# Autodesk Inventor assembly: Zespół1
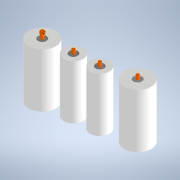
[picture p0: Inventor's stored thumbnail of the model, 180x180]
Saved by Autodesk Inventor 2022 (Build 260153000, 153)
## iProperties
Created: 2023-04-25
Part Number: Zespół1
Document SubType Name: Assembly
Designer: nosal
Author: nosal
## Documents named in this file (6)
- C:\Users\nosal\OneDrive\Pulpit\projekty 3d\Inżynierka\Tasma2\Zespół1.iam
- C:\Users\nosal\OneDrive\Pulpit\projekty 3d\Inżynierka\Tasma2\wał_tylni2.ipt
- C:\Users\nosal\OneDrive\Pulpit\projekty 3d\Inżynierka\Tasma2\wały_sr.ipt
- C:\Users\nosal\OneDrive\Pulpit\projekty 3d\Inżynierka\Tasma2\wal_sr_tyl.ipt
- C:\Users\nosal\OneDrive\Pulpit\projekty 3d\Inżynierka\Tasma2\Design Accelerator\Łożysko1.iam
- C:\Users\nosal\OneDrive\Pulpit\projekty 3d\Inżynierka\Tasma2\wał2.ipt
## Components (16 placed, 5 different names)
1. wał_tylni2:1 — Zestawiające:1, Zestawiające:6, Sztywne:1
2. wał_tylni2:2 — Zestawiające:4, Zestawiające:5, Sztywne:3
3. wały_sr:1 — Zestawiające:2, Zestawiające:7, Sztywne:2
4. wały_sr:2 — Zestawiające:3, Zestawiające:8, Sztywne:4
5. wal_sr_tyl:1 — Sztywne:1
6. Łożysko:1 [sub-assembly] — Zestawiające:2
7. Łożysko:2 [sub-assembly] — Zestawiające:3
8. Łożysko:3 [sub-assembly] — Zestawiające:4
9. Łożysko:4 [sub-assembly] — Zestawiające:5
10. Łożysko:5 [sub-assembly] — Zestawiające:6
11. Łożysko:6 [sub-assembly] — Zestawiające:7
12. Łożysko:7 [sub-assembly] — Zestawiające:8
13. Łożysko:8 [sub-assembly] — Zestawiające:1
14. wał2:1 — Sztywne:4
15. wał2:2 — Sztywne:3
16. wał2:3 — Sztywne:2
## Relationships (12: Mate 8, WeldJoint 4)
- Zestawiające:1 [Mate]: wał_tylni2:1 ↔ Łożysko:8
- Zestawiające:2 [Mate]: wały_sr:1 ↔ Łożysko:1
- Zestawiające:3 [Mate]: wały_sr:2 ↔ Łożysko:2
- Zestawiające:4 [Mate]: wał_tylni2:2 ↔ Łożysko:3
- Zestawiające:5 [Mate]: wał_tylni2:2 ↔ Łożysko:4
- Zestawiające:6 [Mate]: wał_tylni2:1 ↔ Łożysko:5
- Zestawiające:7 [Mate]: wały_sr:1 ↔ Łożysko:6
- Zestawiające:8 [Mate]: wały_sr:2 ↔ Łożysko:7
- Sztywne:1 [WeldJoint] (-150.5 mm): wał_tylni2:1 ↔ wal_sr_tyl:1
- Sztywne:2 [WeldJoint]: wały_sr:1 ↔ wał2:3
- Sztywne:3 [WeldJoint]: wał_tylni2:2 ↔ wał2:2
- Sztywne:4 [WeldJoint]: wały_sr:2 ↔ wał2:1
